# Autodesk Inventor assembly: ETL Module Carrier V1
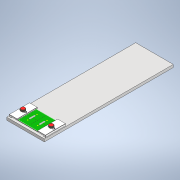
[picture p0: Inventor's stored thumbnail of the model, 180x180]
Saved by Autodesk Inventor 2022 (Build 260153000, 153)
## iProperties
Created: 2022-04-14
Part Number: ETL Module Carrier V1
Document SubType Name: Assembly
Designer: Caleb
Author: Caleb
## Documents named in this file (5)
- C:\Users\Caleb\Desktop\nebraska-silicon-lab\Hardware\ETL\Module Carrier\Module Carrier V1\ETL Module Carrier V1.iam
- C:\Users\Caleb\Desktop\nebraska-silicon-lab\Hardware\ETL\modules\tamale v1.3\Tamale - v1p3.iam
- C:\Users\Caleb\Desktop\nebraska-silicon-lab\Hardware\ETL\Module Carrier\Module Carrier V1\Carrier Plate V1.ipt
- C:\Users\Caleb\Desktop\nebraska-silicon-lab\Hardware\ETL\Module Carrier\Module Carrier V1\Carrier Clip V1.ipt
- C:\Users\Caleb\Desktop\nebraska-silicon-lab\Hardware\ETL\Module Carrier\Module Carrier V1\91185A570_Plastic-Head Thumb Screws.ipt
## Components (6 placed, 4 different names)
1. Tamale - v1p3:1 [sub-assembly] — Mate:1, Angle:1, Cylindrical:1, Cylindrical:2
2. Carrier Plate V1:1 — Mate:1, Angle:1, Mate:2, Angle:2, Mate:3, Angle:3
3. Carrier Clip V1:1 — Mate:2, Angle:2, Cylindrical:1, Mate:4
4. Carrier Clip V1:2 — Mate:3, Angle:3, Cylindrical:2, Mate:5
5. 91185A570_Plastic-Head Thumb Screws:1 — Mate:4
6. 91185A570_Plastic-Head Thumb Screws:2 — Mate:5
## Relationships (10: Mate 5, Angle 3, CylindricalJoint 2)
- Mate:1: Tamale - v1p3:1 ↔ Carrier Plate V1:1
- Angle:1 (0 deg): Tamale - v1p3:1 ↔ Carrier Plate V1:1
- Mate:2: Carrier Plate V1:1 ↔ Carrier Clip V1:1
- Angle:2 (0 deg): Carrier Plate V1:1 ↔ Carrier Clip V1:1
- Cylindrical:1: Tamale - v1p3:1 ↔ Carrier Clip V1:1
- Mate:3: Carrier Plate V1:1 ↔ Carrier Clip V1:2
- Angle:3 (0 deg): Carrier Plate V1:1 ↔ Carrier Clip V1:2
- Cylindrical:2: Tamale - v1p3:1 ↔ Carrier Clip V1:2
- Mate:4: Carrier Clip V1:1 ↔ 91185A570_Plastic-Head Thumb Screws:1
- Mate:5: Carrier Clip V1:2 ↔ 91185A570_Plastic-Head Thumb Screws:2
